# Autodesk Inventor assembly: QLP00ACAB0202#_513.56.511.5
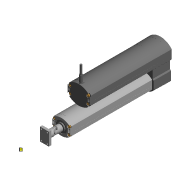
[picture p0: Inventor's stored thumbnail of the model, 180x180]
Saved by Autodesk Inventor 2021 (Build 250183000, 183)
## iProperties
Category: PARTsolutions
Company: ROSEKRIEGER
Part Number: QLP00ACAB0202#_513.56.511.5
Catalog Web Link: www.cadenas.de
Description: Schwerlast-Zylinder LZ 80 mit Trapezgewindespindel-Move-Tec
Vendor: ROSEKRIEGER
Document SubType Name: Assembly
Designer: partserver
Manufacturer: ROSEKRIEGER
Mass: 14309 g
Surface Area: 10199.2 cm^2
Volume: 3374.04 cm^3
Density: 4.24091 g/cm^3
PSOL_IDENT_0: {$CADENAS_DATA\23d-libs\rose_krieger\linearkomponenten\pool_lineartechnik\_hubsaeule_zyliinder\elekt
PSOL_IDENT_1: rozylinder\elekzyl_lz80\elektrozylinder_lz80p_tr_assytable.prj},240 {VTYP=3D},{STYP=ASSTAB},{NB=QLP0
PSOL_IDENT_2: 0ACAB0202#_513.56.511.5},{LINA=QLP00ACAB0202},{NN=Schwerlast-Zylinder LZ 80 mit Trapezgewindespindel
PSOL_IDENT_3: },{DATE=02.12.2020 11:16:39},{GEOMDATE=18.07.2019 09:16:38},{VERSION=},{LINEID=1510},{WBVAR=},{WBNUM
PSOL_IDENT_4: ERIC=}  {NB=QLP00ACAB0202#_513.56.511.5},{LINA=QLP00ACAB0202},{KT=DUMMY},{ARTIKEL=Schwerlast-Zylinde
PSOL_IDENT_5: r},{TYPE=LZ80},{BEST=QLP00ACAB0202},{SPINDEL=TR 24x5},{HINWEINBAUX=Hub + 311 mm},{HUBLAENGE=7.50 mm
PSOL_IDENT_6: bis 397.50 mm},{HUB=202.5},{EINBAUMASSX=513.5},{GEWICHT=14.309},{VORNULL=0},{PPATH=sbl_elektrozylind
PSOL_IDENT_7: er_lz80p_tr.prj},{TEST=202},{YMAXGESCHW=6.5},{YMAXSTROM=11.5},{MAXZUG=C},{IDNR=},{CODE=QLP},{MAXZUGV
PSOL_IDENT_8: IS=10.000 N},{MAXGESCHW=6.5},{MAXSTROM=11.5},{DUMMYDURCH=10.000},{DUMMYLAENG=20.000},{HILFEHUB=105},
PSOL_IDENT_9: {LAENDOPPROFIL=184.500},{RF=1.000},{YHUB=[7.5:397.5/7.5]},{GRUNDKOE=311.000},{YEINBAUMASS=513.5},{EC
PSOL_IDENT_10: LASS80=23-30-18-90},{WARENNUMMER=85011010}
NB: QLP00ACAB0202#_513.56.511.5
NN: Schwerlast-Zylinder LZ 80 mit Trapezgewindespindel
NT: Move-Tec
NBSYN: $BEST.#_$EINBAUMASSX.$MAXGESCHW.$MAXSTROM.
LINA: QLP00ACAB0202
CATALOG: RK Rose+Krieger
ARTIKEL: Schwerlast-Zylinder
TYPE: LZ80
BEST: QLP00ACAB0202
SPINDEL: TR 24x5
HINWEINBAUX: Hub + 311 mm
HUBLAENGE: 7.50 mm bis 397.50 mm
HUB: 202.5
EINBAUMASSX: 513.5
GEWICHT: 14.309
MAXZUGVIS: 10.000 N
MAXGESCHW: 6.5
MAXSTROM: 11.5
ECLASS80: 23-30-18-90
WARENNUMMER: 85011010
SUPPLIER: ROSEKRIEGER
ARTICLENO: QLP00ACAB0202#_513.56.511.5
BOMINFO: QLP00ACAB0202
CREATOR: CADENAS GmbH
Title: QLP00ACAB0202
Author: Cadenas PARTsolutions
Comments: Move-Tec
## Documents named in this file (14)
- C:\Users\Santiago Suárez\Documents\GitHub\Dis.-Mecatronico-E6\inventor proyecto\cilindro\cilindro.iam
- C:\Users\Santiago Suárez\Documents\GitHub\Dis.-Mecatronico-E6\inventor proyecto\cilindro\LZ80_Doppelnutprofil_Hub202_5.ipt
- C:\Users\Santiago Suárez\Documents\GitHub\Dis.-Mecatronico-E6\inventor proyecto\cilindro\LZ80_Gehaeuse_Parallelform.ipt
- C:\Users\Santiago Suárez\Documents\GitHub\Dis.-Mecatronico-E6\inventor proyecto\cilindro\Gehaeusedeckel_Parallelform.ipt
- C:\Users\Santiago Suárez\Documents\GitHub\Dis.-Mecatronico-E6\inventor proyecto\cilindro\Zyl_Schr-M6x30_Stahl_X094085.ipt
- C:\Users\Santiago Suárez\Documents\GitHub\Dis.-Mecatronico-E6\inventor proyecto\cilindro\Funktionsprofil_LZ80.ipt
- C:\Users\Santiago Suárez\Documents\GitHub\Dis.-Mecatronico-E6\inventor proyecto\cilindro\Abdeckkappe_LZ80_funkprofil.ipt
- C:\Users\Santiago Suárez\Documents\GitHub\Dis.-Mecatronico-E6\inventor proyecto\cilindro\Zyl_Schr-M8x30_Stahl_X094960.ipt
- C:\Users\Santiago Suárez\Documents\GitHub\Dis.-Mecatronico-E6\inventor proyecto\cilindro\Abdeckkappe_LZ80.ipt
- C:\Users\Santiago Suárez\Documents\GitHub\Dis.-Mecatronico-E6\inventor proyecto\cilindro\LZ80_Dichtring.ipt
- C:\Users\Santiago Suárez\Documents\GitHub\Dis.-Mecatronico-E6\inventor proyecto\cilindro\LZ80_Zapfen.ipt
- C:\Users\Santiago Suárez\Documents\GitHub\Dis.-Mecatronico-E6\inventor proyecto\cilindro\LZ80_Rohr_Schubstange90.ipt
- C:\Users\Santiago Suárez\Documents\GitHub\Dis.-Mecatronico-E6\inventor proyecto\Cardan\cardan.iam
- C:\Users\Santiago Suárez\Documents\GitHub\Dis.-Mecatronico-E6\inventor proyecto\conector cardan.ipt
## Components (28 placed, 13 different names)
1. LZ80_Doppelnutprofil_Hub202_5:1
2. LZ80_Gehaeuse_Parallelform:1
3. Gehaeusedeckel_Parallelform:1
4. Zyl_Schr-M6x30_Stahl_X094085:1
5. Zyl_Schr-M6x30_Stahl_X094085:2
6. Zyl_Schr-M6x30_Stahl_X094085:3
7. Zyl_Schr-M6x30_Stahl_X094085:4
8. Zyl_Schr-M6x30_Stahl_X094085:5
9. Zyl_Schr-M6x30_Stahl_X094085:6
10. Zyl_Schr-M6x30_Stahl_X094085:7
11. Zyl_Schr-M6x30_Stahl_X094085:8
12. Zyl_Schr-M6x30_Stahl_X094085:9
13. Funktionsprofil_LZ80:1
14. Abdeckkappe_LZ80_funkprofil:1
15. Zyl_Schr-M8x30_Stahl_X094960:1
16. Zyl_Schr-M8x30_Stahl_X094960:2
17. Zyl_Schr-M8x30_Stahl_X094960:3
18. Zyl_Schr-M8x30_Stahl_X094960:4
19. Abdeckkappe_LZ80:1 — Insertar:3
20. LZ80_Dichtring:1
21. Zyl_Schr-M8x30_Stahl_X094960:5
22. Zyl_Schr-M8x30_Stahl_X094960:6
23. Zyl_Schr-M8x30_Stahl_X094960:7
24. Zyl_Schr-M8x30_Stahl_X094960:8
25. LZ80_Zapfen:1 — Rigid:1, Cylindrical:1
26. LZ80_Rohr_Schubstange90:1 — Insertar:3, Cylindrical:1
27. cardan:1 [sub-assembly] — Rigid:1, Mate:1, Insert:4
28. conector cardan:1 — Mate:1, Insert:4
## Relationships (5: Insert 2, WeldJoint 1, CylindricalJoint 1, Mate 1)
- Insertar:3: Abdeckkappe_LZ80:1 ↔ LZ80_Rohr_Schubstange90:1
- Rigid:1 [WeldJoint]: LZ80_Zapfen:1 ↔ cardan:1
- Cylindrical:1: LZ80_Zapfen:1 ↔ LZ80_Rohr_Schubstange90:1
- Mate:1: cardan:1 ↔ conector cardan:1
- Insert:4: cardan:1 ↔ conector cardan:1
